# Autodesk Inventor assembly: Pololu_MotorEncoderModule
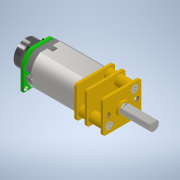
[picture p0: Inventor's stored thumbnail of the model, 180x180]
Saved by Autodesk Inventor 2020 (Build 240168000, 168)
## iProperties
Created: 2020-03-21
Part Number: Pololu_MotorEncoderModule
Document SubType Name: Assembly
Designer: ermoz
Author: ermoz
## Documents named in this file (4)
- D:\Moje Wyczyny\Liceum\VLOat INTvators\Moje projekty\Sneek_100\Electrics Elements\Pololu_MotorEncoderModule.iam
- D:\Moje Wyczyny\Liceum\VLOat INTvators\Moje projekty\Sneek_100\Electrics Elements\Pololu_MicroMotor.ipt
- D:\Moje Wyczyny\Liceum\VLOat INTvators\Moje projekty\Sneek_100\Electrics Elements\Pololu_EncoderMagnes.ipt
- D:\Moje Wyczyny\Liceum\VLOat INTvators\Moje projekty\Sneek_100\Electrics Elements\Pololu_Encoder.ipt
## Components (3 placed, 3 different names)
1. Pololu_MicroMotor:1 — Mate:1, Flush:1, Angle:1, Mate:2, Mate:3
2. Pololu_EncoderMagnes:1 — Mate:1, Flush:1
3. Pololu_Encoder:1 — Angle:1, Mate:2, Mate:3
## Relationships (5: Mate 3, Flush 1, Angle 1)
- Mate:1: Pololu_MicroMotor:1 ↔ Pololu_EncoderMagnes:1
- Flush:1: Pololu_MicroMotor:1 ↔ Pololu_EncoderMagnes:1
- Angle:1 (0 deg): Pololu_MicroMotor:1 ↔ Pololu_Encoder:1
- Mate:2: Pololu_MicroMotor:1 ↔ Pololu_Encoder:1
- Mate:3: Pololu_MicroMotor:1 ↔ Pololu_Encoder:1
